# Autodesk Inventor assembly: Main_assssembly
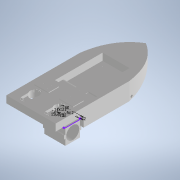
[picture p0: Inventor's stored thumbnail of the model, 180x180]
Saved by Autodesk Inventor 2020.1 (Build 241239000, 239)
## iProperties
Created: 2022-02-07
Part Number: Main_assssembly
Document SubType Name: Assembly
Designer: OEM
Author: OEM
## Documents named in this file (4)
- D:\Studia\Bobr\Repo\CAD\Main_assssembly.iam
- D:\Studia\Bobr\Repo\CAD\MainBody.ipt
- D:\Studia\Bobr\Repo\CAD\connector_sleeve.ipt
- D:\Studia\Bobr\Repo\CAD\engine_sleeve_upper.ipt
## Components (3 placed, 3 different names)
1. MainBody:2 — Rotational:1
2. connector_sleeve:1 — Rotational:1, Mate:1
3. engine_sleeve_upper:1 — Mate:1
## Relationships (2: RevoluteJoint 1, Mate 1)
- Rotational:1 [RevoluteJoint]: MainBody:2 ↔ connector_sleeve:1
- Mate:1: connector_sleeve:1 ↔ engine_sleeve_upper:1
